# Autodesk Inventor assembly: CS2Mazebot
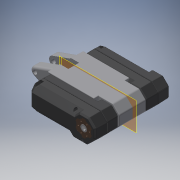
[picture p0: Inventor's stored thumbnail of the model, 180x180]
Saved by Autodesk Inventor 2018 (Build 220112000, 112)
## iProperties
Created: 2018-04-18
Part Number: CS2Mazebot
Document SubType Name: Assembly
Designer: Samuel
Author: Samuel
## Documents named in this file (4)
- C:\Users\Samuel Schuur\Documents\CS2\CS2Mazebot.iam
- C:\Users\Samuel Schuur\Downloads\REV-41-1300.ipt
- C:\Users\Samuel Schuur\Downloads\REV-41-1300_MIR.ipt
- C:\Users\Samuel Schuur\Documents\CS2\ChassisBase.ipt
## Components (3 placed, 3 different names)
1. REV-41-1300:1 — Flush:1, Flush:2
2. REV-41-1300_MIR:1 — Mate:1
3. ChassisBase:1 — Flush:2
## Relationships (3: Flush 2, Mate 1)
- Flush:1 (19.05 mm): REV-41-1300:1
- Mate:1 (19.05 mm): REV-41-1300_MIR:1
- Flush:2: REV-41-1300:1 ↔ ChassisBase:1
